# Autodesk Inventor assembly: AssembledOnLarge
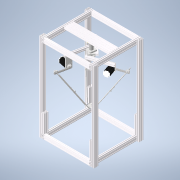
[picture p0: Inventor's stored thumbnail of the model, 180x180]
Saved by Autodesk Inventor 2021 (Build 250183000, 183)
## iProperties
Created: 2022-09-12
Part Number: AssembledOnLarge
Document SubType Name: Assembly
Designer: szucs
Author: szucs
## Documents named in this file (3)
- C:\Users\szucs\Desktop\GTPR\ver2\AssembledOnLarge.iam
- C:\Users\szucs\Desktop\GTPR\ver2\mount\mountLarge.iam
- C:\Users\szucs\Desktop\GTPR\ver2\GTPR Assembly - Laci.iam
## Components (2 placed, 2 different names)
1. mountLarge:1 [sub-assembly] — Mate:1, Mate:2, Mate:3, Angle:1
2. GTPR Assembly - Laci:1 [sub-assembly] — Mate:1, Mate:2, Mate:3, Angle:1
## Relationships (4: Mate 3, Angle 1)
- Mate:1: mountLarge:1 ↔ GTPR Assembly - Laci:1
- Mate:2 (-425 mm): mountLarge:1 ↔ GTPR Assembly - Laci:1
- Mate:3 (-425 mm): mountLarge:1 ↔ GTPR Assembly - Laci:1
- Angle:1 (0 deg): mountLarge:1 ↔ GTPR Assembly - Laci:1
